# Autodesk Inventor assembly: SistemaGeneral
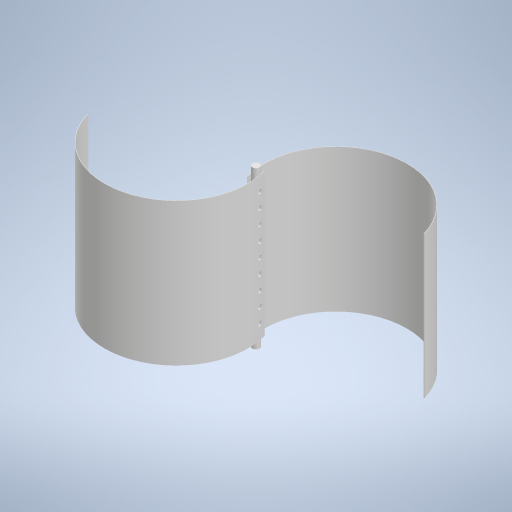
[picture p0: Inventor's stored thumbnail of the model, 512x512]
Saved by Autodesk Inventor 2024 (Build 280153000, 153)
## iProperties
Created: 2024-04-24
Part Number: SistemaGeneral
Document SubType Name: Assembly
Designer: alexa
Author: alexa
## Documents named in this file (3)
- C:\Users\alexa\OneDrive\Escritorio\Energia Eolica\SistemaGeneral.iam
- C:\Users\alexa\OneDrive\Escritorio\Energia Eolica\Aspa.ipt
- C:\Users\alexa\OneDrive\Escritorio\Energia Eolica\EjePrincipal.ipt
## Components (3 placed, 2 different names)
1. EjePrincipal:1 — Mate:1, Flush:1, Mate:2, Mate:3, Mate:4, Mate:5, Mate:6, Mate:7
2. Aspa:1 — Mate:1, Mate:3, Mate:6
3. Aspa:2 — Flush:1, Mate:2, Mate:5
## Relationships (8: Mate 7, Flush 1)
- Mate:1 (-25 mm): EjePrincipal:1 ↔ Aspa:1
- Flush:1 (-25 mm): EjePrincipal:1 ↔ Aspa:2
- Mate:2: EjePrincipal:1 ↔ Aspa:2
- Mate:3: EjePrincipal:1 ↔ Aspa:1
- Mate:4: EjePrincipal:1
- Mate:5: EjePrincipal:1 ↔ Aspa:2
- Mate:6: EjePrincipal:1 ↔ Aspa:1
- Mate:7: EjePrincipal:1
